# Autodesk Inventor assembly: Motor
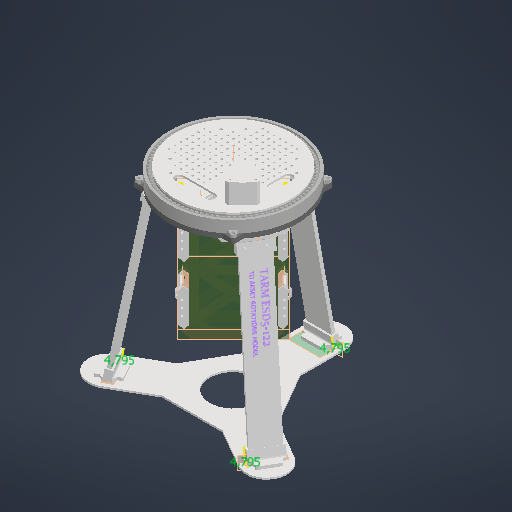
[picture p0: Inventor's stored thumbnail of the model, 512x512]
Saved by Autodesk Inventor 2026.1 (Build 301233020, 233B)
## iProperties
Created: 2025-09-23
Part Number: Motor
Document SubType Name: Assembly
Designer: Malthe Sennels
Author: Malthe Sennels
## Documents named in this file (33)
- C:\Users\Mikke\OneDrive - Aalborg Universitet\ESD 610 - General\Inventor\Base_station\Motor.iam
- C:\Users\Mikke\OneDrive - Aalborg Universitet\ESD 610 - General\Inventor\Base_station\Bearing.ipt
- C:\Users\Mikke\OneDrive - Aalborg Universitet\ESD 610 - General\Inventor\Base_station\Outer_gear.ipt
- C:\Users\Mikke\OneDrive - Aalborg Universitet\ESD 610 - General\Inventor\Base_station\Inner gear.ipt
- C:\Users\Mikke\OneDrive - Aalborg Universitet\ESD 610 - General\Inventor\Base_station\Spur Gears1.iam
- C:\Users\Mikke\OneDrive - Aalborg Universitet\ESD 610 - General\Inventor\Base_station\Venstre arm.ipt
- C:\Users\Mikke\OneDrive - Aalborg Universitet\ESD 610 - General\Inventor\Base_station\Venstre_rotator.ipt
- C:\Users\Mikke\OneDrive - Aalborg Universitet\ESD 610 - General\Inventor\Base_station\Venstre_bearing_lock.ipt
- C:\Users\Mikke\OneDrive - Aalborg Universitet\ESD 610 - General\Inventor\Base_station\Balls.ipt
- C:\Users\Mikke\OneDrive - Aalborg Universitet\ESD 610 - General\Inventor\Base_station\Lazercutlink.ipt
- C:\Users\Mikke\OneDrive - Aalborg Universitet\ESD 610 - General\Inventor\Base_station\Backplane.ipt
- C:\Users\Mikke\OneDrive - Aalborg Universitet\ESD 610 - General\Inventor\Base_station\Lazercut_base.ipt
- C:\Users\Mikke\OneDrive - Aalborg Universitet\ESD 610 - General\Inventor\Base_station\LEG.ipt
- C:\Users\Mikke\OneDrive - Aalborg Universitet\ESD 610 - General\Inventor\Base_station\Lock buttom.ipt
- C:\Users\Mikke\OneDrive - Aalborg Universitet\ESD 610 - General\Inventor\Base_station\Lysekrone_adapter.ipt
- C:\Users\Mikke\OneDrive - Aalborg Universitet\ESD 610 - General\Inventor\Base_station\Center_lysekrone.ipt
- C:\Users\Mikke\OneDrive - Aalborg Universitet\ESD 610 - General\Inventor\Base_station\Krone_interface.ipt
- C:\Users\Mikke\OneDrive - Aalborg Universitet\ESD 610 - General\Inventor\Base_station\Shelf1.ipt
- C:\Users\Mikke\OneDrive - Aalborg Universitet\ESD 610 - General\Inventor\Base_station\Shelf2.ipt
- C:\Users\Mikke\OneDrive - Aalborg Universitet\ESD 610 - General\Inventor\Base_station\RPI_Motordriver_mount.ipt
- C:\Users\Mikke\OneDrive - Aalborg Universitet\ESD 610 - General\Inventor\Base_station\Spacer_1.ipt
- C:\Users\Mikke\OneDrive - Aalborg Universitet\ESD 610 - General\Inventor\Base_station\Spacer_1_MIR.ipt
- C:\Users\Mikke\OneDrive - Aalborg Universitet\ESD 610 - General\Inventor\Base_station\Spacer_1_MIR1.ipt
- C:\Users\Mikke\OneDrive - Aalborg Universitet\ESD 610 - General\Inventor\Base_station\Spacer_1_MIR_MIR.ipt
- C:\Users\Mikke\OneDrive - Aalborg Universitet\ESD 610 - General\Inventor\Base_station\Bund.ipt
- C:\Users\Mikke\OneDrive - Aalborg Universitet\ESD 610 - General\Inventor\Base_station\Pot_holder.ipt
- C:\Users\Mikke\OneDrive - Aalborg Universitet\ESD 610 - General\Inventor\Base_station\Stepper_motor.ipt
- C:\Users\Mikke\OneDrive - Aalborg Universitet\ESD 610 - General\Inventor\Base_station\Stepper_holder.ipt
- C:\Users\Mikke\OneDrive - Aalborg Universitet\ESD 610 - General\Inventor\Base_station\Venstre_rotator_MIR.ipt
- C:\Users\Mikke\OneDrive - Aalborg Universitet\ESD 610 - General\Inventor\Base_station\Stepper_spacer.ipt
- C:\Users\Mikke\OneDrive - Aalborg Universitet\ESD 610 - General\Inventor\Base_station\Motor\Design Accelerator\Spur Gears2.iam
- C:\Users\Mikke\OneDrive - Aalborg Universitet\ESD 610 - General\Inventor\Base_station\Platform.ipt
- C:\Users\Malthe Sennels\OneDrive - Aalborg Universitet\AAUSAT6_CST\Construction\Compass_holder.ipt
## Components (44 placed, 31 different names)
1. Bearing:1 — Flush:2, Flush:3, Flush:7, Flush:8, Mate:2, Flush:21, Flush:22, Flush:23, Flush:24, Flush:30, Mate:7, Mate:8, Mate:9, Flush:41, Mate:26, Mate:27, Mate:28, Mate:29, Mate:30, Flush:68
2. Outer_gear:1 — Flush:3, Flush:37
3. Inner gear:1 — Mate:54
4. Spur Gears:1 [sub-assembly]
5. Venstre arm:1 — Flush:21, Flush:22, Flush:23, Flush:24, Flush:27, Mate:3, Mate:4, Flush:30, Flush:31
6. Venstre_rotator:1 — Mate:4, Flush:31, Mate:17, Mate:18, Mate:19, Flush:65
7. Venstre_bearing_lock:1 — Flush:28, Mate:3
8. Balls:1 — Flush:29
9. Venstre arm:2 — Mate:7, Mate:8, Mate:9, Mate:10, Mate:11, Mate:12, Mate:13, Mate:15, Mate:25, Mate:48, Mate:49, Mate:50, Mate:52
10. Venstre_bearing_lock:2 — Mate:11, Mate:12, Angle:1
11. Balls:2 — Mate:10, Mate:25
12. Lazercutlink:1 — Flush:34
13. Lazercutlink:2 — Mate:17, Mate:18, Mate:19, Mate:24
14. Backplane:1 — Flush:34, Mate:24
15. Lysekrone_adapter:1 — Flush:41, Flush:42, Mate:29, Mate:30
16. Lysekrone_adapter:2 — Mate:26, Mate:27, Mate:28
17. Center_lysekrone:1 — Flush:42, Flush:47, Mate:33, Mate:34, Mate:35, Mate:36
18. Krone_interface:1 — Flush:47, Mate:33, Mate:34, Mate:35, Mate:36, Flush:50, Flush:51
19. Shelf1:1 — Flush:50, Flush:52
20. Shelf2:1 — Flush:51, Flush:53, Flush:54
21. RPI_Motordriver_mount:1 — Flush:52
22. Spacer_1:1 — Flush:53, Flush:54, Flush:66
23. Spacer_1_MIR:1
24. Spacer_1_MIR1:1
25. Spacer_1_MIR_MIR:1
26. Bund:1 — Flush:63, Flush:64, Mate:44
27. Pot_holder:1 — Flush:65
28. Stepper_motor:1 — Mate:53, Mate:54, Mate:55, Mate:56
29. Stepper_holder:1 — Flush:66
30. Stepper_motor:2 — Flush:67, Mate:48, Mate:50, Mate:51
31. Venstre_rotator_MIR:1
32. Stepper_spacer:1 — Flush:67, Mate:49
33. Spur Gears:2 [sub-assembly] — Mate:51, Mate:52
34. Platform:1 — Flush:68, Mate:53, Mate:55, Mate:56, Flush:69, Flush:70
35. Compass_holder:1 — Flush:69, Flush:70
36. Lazercut_base:1 — Flush:37
37. Lazercut_base:2 — Flush:38
38. Lazercut_base:3
39. LEG:1 — Flush:38
40. LEG:2
41. LEG:3 — Flush:39, Mate:45, Mate:46
42. Lock buttom:1 — Mate:44, Mate:45, Mate:46
43. Lock buttom:2
44. Lock buttom:3
## Component patterns: (3 elements, first: Lazercut_base:1), (3 elements, first: LEG:1), (3 elements, first: Lock buttom:1)
## Relationships (73: Mate 38, Flush 33, Angle 2)
- Flush:2: Bearing:1
- Flush:3 (3 mm): Bearing:1 ↔ Outer_gear:1
- Flush:7 (-8 mm): Bearing:1
- Flush:8: Bearing:1
- Mate:2: Bearing:1
- Flush:21: Bearing:1 ↔ Venstre arm:1
- Flush:22: Bearing:1 ↔ Venstre arm:1
- Flush:23: Bearing:1 ↔ Venstre arm:1
- Flush:24: Bearing:1 ↔ Venstre arm:1
- Flush:27 (0.15 mm): Venstre arm:1
- Flush:28: Venstre_bearing_lock:1
- Mate:3: Venstre arm:1 ↔ Venstre_bearing_lock:1
- Flush:29: Balls:1
- Mate:4: Venstre arm:1 ↔ Venstre_rotator:1
- Flush:30: Bearing:1 ↔ Venstre arm:1
- [Mate]: Venstre arm:2 ↔ Venstre_bearing_lock:2
- Mate:7: Bearing:1 ↔ Venstre arm:2
- Mate:8: Bearing:1 ↔ Venstre arm:2
- Mate:9: Bearing:1 ↔ Venstre arm:2
- Mate:10: Venstre arm:2 ↔ Balls:2
- Mate:11: Venstre arm:2 ↔ Venstre_bearing_lock:2
- Mate:12: Venstre arm:2 ↔ Venstre_bearing_lock:2
- Flush:31: Venstre arm:1 ↔ Venstre_rotator:1
- Mate:13: Venstre arm:2
- Angle:1 (90 deg): Venstre_bearing_lock:2
- Mate:15: Venstre arm:2
- Angle:2 (90 deg)
- Mate:17: Venstre_rotator:1 ↔ Lazercutlink:2
- Mate:18: Venstre_rotator:1 ↔ Lazercutlink:2
- Mate:19: Venstre_rotator:1 ↔ Lazercutlink:2
- Flush:34: Lazercutlink:1 ↔ Backplane:1
- Flush:37: Outer_gear:1 ↔ Lazercut_base:1
- Flush:38: Lazercut_base:2 ↔ LEG:1
- Flush:39 (-60 mm): LEG:3
- Mate:24: Lazercutlink:2 ↔ Backplane:1
- Mate:25: Venstre arm:2 ↔ Balls:2
- Flush:41: Bearing:1 ↔ Lysekrone_adapter:1
- Mate:26: Bearing:1 ↔ Lysekrone_adapter:2
- Mate:27: Bearing:1 ↔ Lysekrone_adapter:2
- Mate:28: Bearing:1 ↔ Lysekrone_adapter:2
- Flush:42: Lysekrone_adapter:1 ↔ Center_lysekrone:1
- Mate:29: Bearing:1 ↔ Lysekrone_adapter:1
- Mate:30: Bearing:1 ↔ Lysekrone_adapter:1
- Flush:47: Center_lysekrone:1 ↔ Krone_interface:1
- Mate:33: Center_lysekrone:1 ↔ Krone_interface:1
- Mate:34: Center_lysekrone:1 ↔ Krone_interface:1
- Mate:35: Center_lysekrone:1 ↔ Krone_interface:1
- Mate:36: Center_lysekrone:1 ↔ Krone_interface:1
- Flush:50: Krone_interface:1 ↔ Shelf1:1
- Flush:51: Krone_interface:1 ↔ Shelf2:1
- Flush:52: Shelf1:1 ↔ RPI_Motordriver_mount:1
- Flush:53: Shelf2:1 ↔ Spacer_1:1
- Flush:54: Shelf2:1 ↔ Spacer_1:1
- Flush:63: Bund:1
- Flush:64: Bund:1
- Mate:44: Bund:1 ↔ Lock buttom:1
- Mate:45: LEG:3 ↔ Lock buttom:1
- Mate:46: LEG:3 ↔ Lock buttom:1
- Flush:65: Venstre_rotator:1 ↔ Pot_holder:1
- Flush:66: Spacer_1:1 ↔ Stepper_holder:1
- Flush:67: Stepper_motor:2 ↔ Stepper_spacer:1
- Mate:48: Venstre arm:2 ↔ Stepper_motor:2
- Mate:49: Venstre arm:2 ↔ Stepper_spacer:1
- Mate:50: Venstre arm:2 ↔ Stepper_motor:2
- Mate:51: Stepper_motor:2 ↔ Spur Gears:2
- Mate:52: Venstre arm:2 ↔ Spur Gears:2
- Flush:68: Bearing:1 ↔ Platform:1
- Mate:53: Stepper_motor:1 ↔ Platform:1
- Mate:54: Inner gear:1 ↔ Stepper_motor:1
- Mate:55: Stepper_motor:1 ↔ Platform:1
- Mate:56: Stepper_motor:1 ↔ Platform:1
- Flush:69: Platform:1 ↔ Compass_holder:1
- Flush:70: Platform:1 ↔ Compass_holder:1
## Named parameters: d48_d43 = 0 mm
